# Autodesk Inventor assembly: TempController
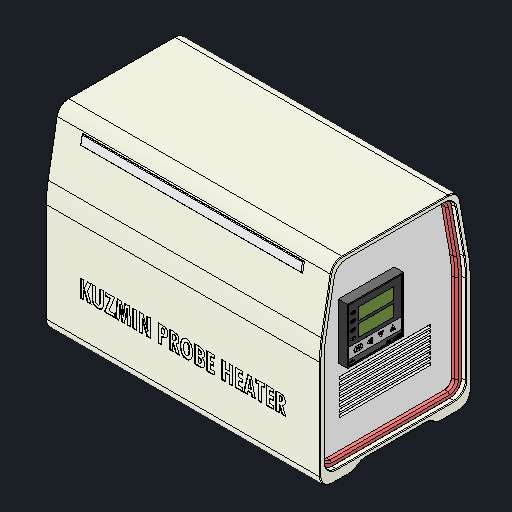
[picture p0: Inventor's stored thumbnail of the model, 512x512]
Saved by Autodesk Inventor 2027.1 (Build 311270010, 270A)
## iProperties
Created: 2025-05-30
Part Number: TempController
Document SubType Name: Assembly
Designer: kuzmin
Author: kuzmin
## Documents named in this file (25)
- C:\Users\queezz\Dropbox\Drawings\PIHTI\ElectronicsBox\TempController-v2\TempController-v2.iam
- C:\Users\queezz\Dropbox\Drawings\PIHTI\ElectronicsBox\TempController-v2\RKC CONTROLLER v2.ipt
- C:\Users\queezz\Dropbox\Drawings\PIHTI\ElectronicsBox\TempController-v2\tc-front-panel-150W.ipt
- C:\Users\queezz\Dropbox\Drawings\PIHTI\ElectronicsBox\TempController\Wide Din Clip V1.ipt
- C:\Users\queezz\Dropbox\Drawings\PIHTI\ElectronicsBox\TempController\DIN-rail-tc.ipt
- C:\Users\queezz\Dropbox\Drawings\PIHTI\ElectronicsBox\TempController-v2\tc-bottom-tray-150W.ipt
- C:\Users\queezz\Dropbox\Drawings\PIHTI\ElectronicsBox\TempController-v2\SSR-on-DIN.iam
- C:\Users\queezz\Dropbox\Drawings\PIHTI\ElectronicsBox\TempController\IEC320 C14 Panel switch.ipt
- C:\Users\queezz\Dropbox\Drawings\PIHTI\ElectronicsBox\TempController-v2\tc-back-panel-150W.ipt
- C:\Users\queezz\Dropbox\Drawings\PIHTI\ElectronicsBox\TempController-v2\tc-case-150W.ipt
- C:\Users\queezz\Dropbox\Drawings\PIHTI\ElectronicsBox\TempController-v2\tc-top-bar-150W.ipt
- C:\Users\queezz\Dropbox\Drawings\PIHTI\ContentCenter\Fastners\M3x16-SHCS.ipt
- C:\Users\queezz\Dropbox\Drawings\PIHTI\ContentCenter\Fastners\M3-nut.ipt
- C:\Users\queezz\Dropbox\Drawings\PIHTI\ElectronicsBox\TempController-v2\STEPs\Type-K Thermocouple Mini Socket\Type-K Thermocouple Mini Socket.iam
- C:\Users\queezz\Dropbox\Drawings\PIHTI\ElectronicsBox\TempController-v2\Wago-3x3.ipt
- C:\Users\queezz\Dropbox\Drawings\PIHTI\ContentCenter\Fastners\M3x10-SHCS.ipt
- C:\Users\queezz\Dropbox\Drawings\PIHTI\ElectronicsBox\TempController-v2\40x40x10 DC Fan.ipt
- C:\Users\queezz\Dropbox\Drawings\PIHTI\ContentCenter\Fastners\brass-insert-m3x5.ipt
- C:\Users\queezz\Dropbox\Drawings\PIHTI\ContentCenter\Electrics\Amass_XT60E-F.iam
- C:\Users\queezz\Dropbox\Drawings\PIHTI\ContentCenter\Fastners\M3x8-countersunk.ipt
- C:\Users\queezz\Dropbox\Drawings\PIHTI\ElectronicsBox\TempController-v2\fan-holder.ipt
- C:\Users\queezz\Dropbox\Drawings\PIHTI\ContentCenter\Fastners\M3x8-SHCS.ipt
- C:\Users\queezz\Dropbox\Drawings\PIHTI\ContentCenter\Fastners\M3x12-SHCS.ipt
- C:\Users\queezz\Dropbox\Drawings\PIHTI\ElectronicsBox\TempController-v2\LRS-150.ipt
- C:\Users\queezz\Dropbox\Drawings\PIHTI\ElectronicsBox\TempController-v2\LRS-150-din-bracket.ipt
## Components (52 placed, 24 different names)
1. tc-front-panel-150W:1 — Mate:1, Mate:2, Mate:3, Mate:7, Flush:1, Flush:3, Flush:4, Flush:5, Flush:6, Mate:14, Flush:8, Rigid:7, Rigid:8, Rigid:9, Rigid:10
2. RKC CONTROLLER v2:1 — Mate:1, Mate:2, Mate:3
3. Wide Din Clip V1:1 — Mate:4, Mate:5, Rigid:46
4. DIN-rail-tc:1 — Mate:4, Mate:5, Mate:6, Flush:2, Mate:8, Mate:9
5. tc-bottom-tray-150W:1 — Mate:6, Mate:7, Flush:1, Flush:2, Flush:3, Mate:10, Rigid:19, Rigid:20, Rigid:21, Rigid:22, Rigid:23, Rigid:26, Rigid:27
6. SSR-on-DIN:1 [sub-assembly] — Mate:8, Mate:9
7. IEC320 C14 Panel switch:1 — Rotational:1, Rigid:35, Rigid:36
8. tc-back-panel-150W:1 — Flush:4, Flush:5, Mate:10, Mate:15, Mate:16, Flush:9, Rigid:15, Rigid:16, Rigid:17, Rigid:18, Rotational:1, Rigid:28, Rigid:29, Rotational:2, Rotational:3, Mate:25, Mate:26, Mate:27, Mate:28, Mate:29, Mate:30, Rigid:49, Rigid:50
9. tc-case-150W:1 — Flush:6, Mate:14, Mate:15
10. tc-top-bar-150W:1 — Mate:16, Flush:7, Flush:9, Rigid:11, Rigid:12, Rigid:13, Rigid:14
11. Type-K Thermocouple Mini Socket:1 [sub-assembly] — Mate:25, Mate:26, Mate:27
12. Type-K Thermocouple Mini Socket:2 [sub-assembly] — Mate:28, Mate:29, Mate:30
13. Wago-3x3:1 — Rigid:23, Rigid:24, Rigid:25
14. 40x40x10 DC Fan:1 — Rigid:38, Rigid:42, Rigid:43, Rigid:44, Rigid:45
15. Amass_XT60E-F:1 [sub-assembly] — Rigid:33, Rigid:34, Rigid:50
16. fan-holder:1 — Rigid:38, Rigid:40, Rigid:41, Rigid:49
17. LRS-150:1 — Rigid:47
18. LRS-150-din-bracket:1 — Rigid:46, Rigid:47
19. AS 1420 - Metric M3 x 12:1 — Rigid:44
20. AS 1420 - Metric M3 x 12:2 — Rigid:43
21. AS 1420 - Metric M3 x 12:3 — Rigid:42
22. AS 1420 - Metric M3 x 12:4 — Rigid:45
23. SS ISO 4762 M3 x 8:1 — Rigid:40
24. SS ISO 4762 M3 x 8:2 — Rigid:41
25. brass-insert-m3x5:1 — Rigid:28
26. brass-insert-m3x5:2 — Rigid:29
27. JIS B 1181 Style 1 - Metric A M3:9 — Rigid:26
28. JIS B 1181 Style 1 - Metric A M3:10 — Rigid:27
29. brass-insert-m3x5:4 — Rotational:3
30. brass-insert-m3x5:3 — Rotational:2
31. UNI 5933 M3 x 8:1 — Rigid:34
32. UNI 5933 M3 x 8:2 — Rigid:36
33. UNI 5933 M3 x 8:3 — Rigid:35
34. UNI 5933 M3 x 8:4 — Rigid:33
35. JIS B 1176 - Metric M3 x 10:1 — Rigid:24
36. JIS B 1176 - Metric M3 x 10:2 — Rigid:25
37. JIS B 1181 Style 1 - Metric A M3:5 — Rigid:18
38. JIS B 1181 Style 1 - Metric A M3:6 — Rigid:16
39. JIS B 1181 Style 1 - Metric A M3:7 — Rigid:17
40. JIS B 1181 Style 1 - Metric A M3:8 — Rigid:15
41. SS ISO 4762 M3 x 16:1 — Rigid:21
42. SS ISO 4762 M3 x 16:2 — Rigid:22
43. SS ISO 4762 M3 x 16:3 — Rigid:19
44. SS ISO 4762 M3 x 16:4 — Rigid:20
45. JIS B 1181 Style 1 - Metric A M3:1 — Rigid:9
46. JIS B 1181 Style 1 - Metric A M3:2 — Rigid:10
47. JIS B 1181 Style 1 - Metric A M3:3 — Rigid:8
48. JIS B 1181 Style 1 - Metric A M3:4 — Rigid:7
49. SS ISO 4762 M3 x 16:5 — Rigid:12
50. SS ISO 4762 M3 x 16:6 — Rigid:11
51. SS ISO 4762 M3 x 16:7 — Rigid:14
52. SS ISO 4762 M3 x 16:8 — Rigid:13
## Relationships (69: WeldJoint 38, Mate 19, Flush 9, RevoluteJoint 3)
- Mate:1: tc-front-panel-150W:1 ↔ RKC CONTROLLER v2:1
- Mate:2: tc-front-panel-150W:1 ↔ RKC CONTROLLER v2:1
- Mate:3: tc-front-panel-150W:1 ↔ RKC CONTROLLER v2:1
- Mate:4: Wide Din Clip V1:1 ↔ DIN-rail-tc:1
- Mate:5: Wide Din Clip V1:1 ↔ DIN-rail-tc:1
- Mate:6: DIN-rail-tc:1 ↔ tc-bottom-tray-150W:1
- Mate:7: tc-front-panel-150W:1 ↔ tc-bottom-tray-150W:1
- Flush:1: tc-front-panel-150W:1 ↔ tc-bottom-tray-150W:1
- Flush:2: DIN-rail-tc:1 ↔ tc-bottom-tray-150W:1
- Flush:3 (5 mm): tc-front-panel-150W:1 ↔ tc-bottom-tray-150W:1
- Mate:8: DIN-rail-tc:1 ↔ SSR-on-DIN:1
- Mate:9: DIN-rail-tc:1 ↔ SSR-on-DIN:1
- Flush:4: tc-front-panel-150W:1 ↔ tc-back-panel-150W:1
- Flush:5: tc-front-panel-150W:1 ↔ tc-back-panel-150W:1
- Mate:10: tc-bottom-tray-150W:1 ↔ tc-back-panel-150W:1
- Flush:6: tc-front-panel-150W:1 ↔ tc-case-150W:1
- Mate:14: tc-front-panel-150W:1 ↔ tc-case-150W:1
- Mate:15: tc-back-panel-150W:1 ↔ tc-case-150W:1
- Mate:16: tc-back-panel-150W:1 ↔ tc-top-bar-150W:1
- Flush:7: tc-top-bar-150W:1
- Flush:8: tc-front-panel-150W:1
- Flush:9 (2 mm): tc-back-panel-150W:1 ↔ tc-top-bar-150W:1
- Rigid:7 [WeldJoint]: tc-front-panel-150W:1 ↔ JIS B 1181 Style 1 - Metric A M3:4
- Rigid:8 [WeldJoint]: tc-front-panel-150W:1 ↔ JIS B 1181 Style 1 - Metric A M3:3
- Rigid:9 [WeldJoint]: tc-front-panel-150W:1 ↔ JIS B 1181 Style 1 - Metric A M3:1
- Rigid:10 [WeldJoint]: tc-front-panel-150W:1 ↔ JIS B 1181 Style 1 - Metric A M3:2
- Rigid:11 [WeldJoint]: tc-top-bar-150W:1 ↔ SS ISO 4762 M3 x 16:6
- Rigid:12 [WeldJoint]: tc-top-bar-150W:1 ↔ SS ISO 4762 M3 x 16:5
- Rigid:13 [WeldJoint]: tc-top-bar-150W:1 ↔ SS ISO 4762 M3 x 16:8
- Rigid:14 [WeldJoint]: tc-top-bar-150W:1 ↔ SS ISO 4762 M3 x 16:7
- Rigid:15 [WeldJoint]: tc-back-panel-150W:1 ↔ JIS B 1181 Style 1 - Metric A M3:8
- Rigid:16 [WeldJoint]: tc-back-panel-150W:1 ↔ JIS B 1181 Style 1 - Metric A M3:6
- Rigid:17 [WeldJoint]: tc-back-panel-150W:1 ↔ JIS B 1181 Style 1 - Metric A M3:7
- Rigid:18 [WeldJoint]: tc-back-panel-150W:1 ↔ JIS B 1181 Style 1 - Metric A M3:5
- Rigid:19 [WeldJoint]: tc-bottom-tray-150W:1 ↔ SS ISO 4762 M3 x 16:3
- Rigid:20 [WeldJoint]: tc-bottom-tray-150W:1 ↔ SS ISO 4762 M3 x 16:4
- Rigid:21 [WeldJoint]: tc-bottom-tray-150W:1 ↔ SS ISO 4762 M3 x 16:1
- Rigid:22 [WeldJoint]: tc-bottom-tray-150W:1 ↔ SS ISO 4762 M3 x 16:2
- Rigid:23 [WeldJoint]: tc-bottom-tray-150W:1 ↔ Wago-3x3:1
- Rigid:24 [WeldJoint]: Wago-3x3:1 ↔ JIS B 1176 - Metric M3 x 10:1
- Rigid:25 [WeldJoint]: Wago-3x3:1 ↔ JIS B 1176 - Metric M3 x 10:2
- Rigid:26 [WeldJoint]: tc-bottom-tray-150W:1 ↔ JIS B 1181 Style 1 - Metric A M3:9
- Rigid:27 [WeldJoint]: tc-bottom-tray-150W:1 ↔ JIS B 1181 Style 1 - Metric A M3:10
- Rotational:1 [RevoluteJoint]: IEC320 C14 Panel switch:1 ↔ tc-back-panel-150W:1
- Rigid:28 [WeldJoint]: tc-back-panel-150W:1 ↔ brass-insert-m3x5:1
- Rigid:29 [WeldJoint]: tc-back-panel-150W:1 ↔ brass-insert-m3x5:2
- Rotational:2 [RevoluteJoint]: tc-back-panel-150W:1 ↔ brass-insert-m3x5:3
- Rotational:3 [RevoluteJoint]: tc-back-panel-150W:1 ↔ brass-insert-m3x5:4
- Rigid:33 [WeldJoint]: Amass_XT60E-F:1 ↔ UNI 5933 M3 x 8:4
- Rigid:34 [WeldJoint]: Amass_XT60E-F:1 ↔ UNI 5933 M3 x 8:1
- Rigid:35 [WeldJoint]: IEC320 C14 Panel switch:1 ↔ UNI 5933 M3 x 8:3
- Rigid:36 [WeldJoint]: IEC320 C14 Panel switch:1 ↔ UNI 5933 M3 x 8:2
- Rigid:38 [WeldJoint]: 40x40x10 DC Fan:1 ↔ fan-holder:1
- Rigid:40 [WeldJoint]: fan-holder:1 ↔ SS ISO 4762 M3 x 8:1
- Rigid:41 [WeldJoint]: fan-holder:1 ↔ SS ISO 4762 M3 x 8:2
- Rigid:42 [WeldJoint]: 40x40x10 DC Fan:1 ↔ AS 1420 - Metric M3 x 12:3
- Rigid:43 [WeldJoint]: 40x40x10 DC Fan:1 ↔ AS 1420 - Metric M3 x 12:2
- Rigid:44 [WeldJoint]: 40x40x10 DC Fan:1 ↔ AS 1420 - Metric M3 x 12:1
- Rigid:45 [WeldJoint]: 40x40x10 DC Fan:1 ↔ AS 1420 - Metric M3 x 12:4
- Rigid:46 [WeldJoint]: Wide Din Clip V1:1 ↔ LRS-150-din-bracket:1
- Rigid:47 [WeldJoint]: LRS-150:1 ↔ LRS-150-din-bracket:1
- Mate:25: tc-back-panel-150W:1 ↔ Type-K Thermocouple Mini Socket:1
- Mate:26: tc-back-panel-150W:1 ↔ Type-K Thermocouple Mini Socket:1
- Mate:27: tc-back-panel-150W:1 ↔ Type-K Thermocouple Mini Socket:1
- Mate:28: tc-back-panel-150W:1 ↔ Type-K Thermocouple Mini Socket:2
- Mate:29: tc-back-panel-150W:1 ↔ Type-K Thermocouple Mini Socket:2
- Mate:30: tc-back-panel-150W:1 ↔ Type-K Thermocouple Mini Socket:2
- Rigid:49 [WeldJoint]: tc-back-panel-150W:1 ↔ fan-holder:1
- Rigid:50 [WeldJoint] (0.6 mm): tc-back-panel-150W:1 ↔ Amass_XT60E-F:1
## Named parameters: insert_width = 1 mm, insert_hight = 1 mm, insert_length = 180 mm
